# Autodesk Inventor assembly: arm
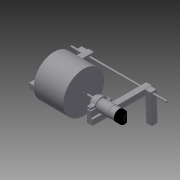
[picture p0: Inventor's stored thumbnail of the model, 180x180]
Saved by Autodesk Inventor 2015 (Build 190159000, 159)
## iProperties
Created: 2014-10-11
Part Number: arm
Document SubType Name: Assembly
Designer: jesse
Author: jesse
## Documents named in this file (8)
- C:\Users\jesse\Desktop\robot\arm\arm.iam
- C:\Users\jesse\Desktop\robot\arm\sidepeices.ipt
- C:\Users\jesse\Desktop\robot\stock parts\dc_motor_mount_2012\dc_motor_mount_2012.ipt
- C:\Users\jesse\Desktop\robot\arm\other side roller axle holder.ipt
- C:\Users\jesse\Desktop\robot\arm\arm axle.ipt
- C:\Users\jesse\Desktop\robot\roller.ipt
- C:\Users\jesse\Desktop\robot\stock parts\am-2964NeveRest\am-2964NeveRest.ipt
- C:\Users\jesse\Desktop\robot\arm\arm holder mount thing.ipt
## Components (9 placed, 7 different names)
1. sidepeices:1 — Flush:1, Flush:2, Flush:3, Mate:2, Flush:4, Mate:4, Mate:10
2. sidepeices:2 — Flush:1, Flush:2, Mate:3, Flush:6, Mate:8, Mate:12
3. dc_motor_mount_2012:1 — Flush:3, Mate:2, Flush:4, Mate:6
4. other side roller axle holder:1 — Mate:3, Flush:6, Mate:5, Mate:8
5. arm axle:1 — Mate:4, Mate:9, Mate:11
6. roller:1 — Mate:5, Mate:7
7. am-2964NeveRest:1 — Mate:6, Mate:7
8. arm holder mount thing:1 — Mate:9, Mate:10, Flush:7
9. arm holder mount thing:2 — Mate:11, Mate:12, Flush:7
## Relationships (17: Mate 11, Flush 6)
- Flush:1: sidepeices:1 ↔ sidepeices:2
- Flush:2: sidepeices:1 ↔ sidepeices:2
- Flush:3: sidepeices:1 ↔ dc_motor_mount_2012:1
- Mate:2: sidepeices:1 ↔ dc_motor_mount_2012:1
- Flush:4: sidepeices:1 ↔ dc_motor_mount_2012:1
- Mate:3: sidepeices:2 ↔ other side roller axle holder:1
- Flush:6: sidepeices:2 ↔ other side roller axle holder:1
- Mate:4: sidepeices:1 ↔ arm axle:1
- Mate:5: other side roller axle holder:1 ↔ roller:1
- Mate:6: dc_motor_mount_2012:1 ↔ am-2964NeveRest:1
- Mate:7: roller:1 ↔ am-2964NeveRest:1
- Mate:8: sidepeices:2 ↔ other side roller axle holder:1
- Mate:9: arm axle:1 ↔ arm holder mount thing:1
- Mate:10: sidepeices:1 ↔ arm holder mount thing:1
- Mate:11: arm axle:1 ↔ arm holder mount thing:2
- Mate:12: sidepeices:2 ↔ arm holder mount thing:2
- Flush:7: arm holder mount thing:1 ↔ arm holder mount thing:2
